# Autodesk Inventor assembly: intake
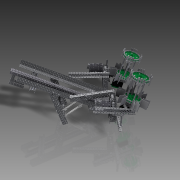
[picture p0: Inventor's stored thumbnail of the model, 180x180]
Saved by Autodesk Inventor 2014 SP1 (Build 180222100, 222)
## iProperties
Created: 2014-02-27
Part Number: intake
Document SubType Name: Assembly
Designer: Ryan
Author: Ryan
## Documents named in this file (6)
- C:\Users\Ryan\Desktop\sw\toss up 4th robot\intake\intake.iam
- C:\Users\Ryan\Desktop\sw\toss up 4th robot\intake\spinning thing.iam
- C:\Users\Ryan\Desktop\sw\toss up 4th robot\intake\intake part on end of six bar.iam
- C:\Users\Ryan\Desktop\sw\toss up 4th robot\intake\sled.iam
- C:\Users\Ryan\Desktop\sw\lib\Aperture VEX CAD Library\Spacers\SPACER-0500-0125.ipt
- C:\Users\Ryan\Desktop\sw\toss up 4th robot\intake\intake part on end of six bar_MIR.iam
## Components (15 placed, 5 different names)
1. spinning thing:1 [sub-assembly] — Mate:1, Mate:2
2. intake part on end of six bar:1 [sub-assembly] — Mate:1, Mate:2, Mate:3, Mate:5, Mate:7, Mate:12, Mate:13, Mate:14, Mate:22, Mate:25, Mate:39, Mate:40
3. sled:1 [sub-assembly] — Mate:3, Mate:5, Mate:8, Mate:9, Mate:23, Mate:27, Mate:30, Mate:37
4. SPACER-0500-0125:1 — Mate:7, Mate:8, Mate:9, Mate:21, Mate:23, Mate:29
5. intake part on end of six bar_MIR:1 [sub-assembly] — Mate:10, Mate:11, Mate:12, Mate:13, Mate:14, Mate:17, Mate:26, Mate:38, Mate:41
6. spinning thing:2 [sub-assembly] — Mate:10, Mate:11
7. SPACER-0500-0125:2 — Mate:17, Mate:18, Mate:19, Mate:33, Mate:34
8. SPACER-0500-0125:3 — Mate:18, Mate:19, Mate:38
9. SPACER-0500-0125:4 — Mate:21, Mate:22, Mate:39
10. SPACER-0500-0125:5 — Mate:25, Mate:31, Mate:40
11. SPACER-0500-0125:6 — Mate:26, Mate:27, Mate:35, Mate:36
12. SPACER-0500-0125:7 — Mate:29
13. SPACER-0500-0125:8 — Mate:30, Mate:31
14. SPACER-0500-0125:9 — Mate:33, Mate:34, Mate:37
15. SPACER-0500-0125:10 — Mate:35, Mate:36
## Relationships (33: Mate 33)
- Mate:1: spinning thing:1 ↔ intake part on end of six bar:1
- Mate:2: spinning thing:1 ↔ intake part on end of six bar:1
- Mate:3 (2.3114 mm): intake part on end of six bar:1 ↔ sled:1
- Mate:5 (2.3114 mm): intake part on end of six bar:1 ↔ sled:1
- Mate:7: intake part on end of six bar:1 ↔ SPACER-0500-0125:1
- Mate:8 (2.3114 mm): sled:1 ↔ SPACER-0500-0125:1
- Mate:9 (2.3114 mm): sled:1 ↔ SPACER-0500-0125:1
- Mate:10: intake part on end of six bar_MIR:1 ↔ spinning thing:2
- Mate:11: intake part on end of six bar_MIR:1 ↔ spinning thing:2
- Mate:12: intake part on end of six bar:1 ↔ intake part on end of six bar_MIR:1
- Mate:13: intake part on end of six bar:1 ↔ intake part on end of six bar_MIR:1
- Mate:14: intake part on end of six bar:1 ↔ intake part on end of six bar_MIR:1
- Mate:17: intake part on end of six bar_MIR:1 ↔ SPACER-0500-0125:2
- Mate:18: SPACER-0500-0125:2 ↔ SPACER-0500-0125:3
- Mate:19: SPACER-0500-0125:2 ↔ SPACER-0500-0125:3
- Mate:21: SPACER-0500-0125:1 ↔ SPACER-0500-0125:4
- Mate:22: intake part on end of six bar:1 ↔ SPACER-0500-0125:4
- Mate:23 (3.175 mm): sled:1 ↔ SPACER-0500-0125:1
- Mate:25: intake part on end of six bar:1 ↔ SPACER-0500-0125:5
- Mate:26: intake part on end of six bar_MIR:1 ↔ SPACER-0500-0125:6
- Mate:27: sled:1 ↔ SPACER-0500-0125:6
- Mate:29: SPACER-0500-0125:1 ↔ SPACER-0500-0125:7
- Mate:30: sled:1 ↔ SPACER-0500-0125:8
- Mate:31: SPACER-0500-0125:5 ↔ SPACER-0500-0125:8
- Mate:33: SPACER-0500-0125:2 ↔ SPACER-0500-0125:9
- Mate:34: SPACER-0500-0125:2 ↔ SPACER-0500-0125:9
- Mate:35: SPACER-0500-0125:6 ↔ SPACER-0500-0125:10
- Mate:36: SPACER-0500-0125:6 ↔ SPACER-0500-0125:10
- Mate:37: sled:1 ↔ SPACER-0500-0125:9
- Mate:38: intake part on end of six bar_MIR:1 ↔ SPACER-0500-0125:3
- Mate:39: intake part on end of six bar:1 ↔ SPACER-0500-0125:4
- Mate:40: intake part on end of six bar:1 ↔ SPACER-0500-0125:5
- Mate:41: intake part on end of six bar_MIR:1
## Named parameters: q = 2.3114 mm
